# Autodesk Inventor assembly: RackPinionTest
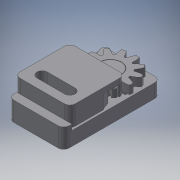
[picture p0: Inventor's stored thumbnail of the model, 180x180]
Saved by Autodesk Inventor 2019 (Build 230136000, 136)
## iProperties
Created: 2019-08-06
Part Number: RackPinionTest
Document SubType Name: Assembly
Designer: aorfi
Author: aorfi
## Documents named in this file (5)
- C:\Users\aorfi\Documents\IQC\CustomParts\RackPinionTest.iam
- C:\Users\aorfi\Documents\IQC\CustomParts\PinionHolderTest.ipt
- C:\Users\aorfi\Documents\IQC\CustomParts\Pinion.ipt
- C:\Users\aorfi\Documents\IQC\CustomParts\Pawl.ipt
- C:\Users\aorfi\Documents\IQC\CustomParts\RackTest.ipt
## Components (4 placed, 4 different names)
1. PinionHolderTest:1 — Mate:1, Mate:2, Flush:1, Mate:3, Mate:4, Mate:5, Mate:6, Mate:8, Mate:9
2. Pinion:1 — Mate:5, Mate:6
3. Pawl:1 — Mate:3, Mate:4
4. RackTest:1 — Mate:8, Mate:9
## Relationships (9: Mate 8, Flush 1)
- Mate:1: PinionHolderTest:1
- Mate:2: PinionHolderTest:1
- Flush:1: PinionHolderTest:1
- Mate:3: PinionHolderTest:1 ↔ Pawl:1
- Mate:4: PinionHolderTest:1 ↔ Pawl:1
- Mate:5: PinionHolderTest:1 ↔ Pinion:1
- Mate:6: PinionHolderTest:1 ↔ Pinion:1
- Mate:8: PinionHolderTest:1 ↔ RackTest:1
- Mate:9: PinionHolderTest:1 ↔ RackTest:1
